# Autodesk Inventor assembly: XY Joint-Unit [B]
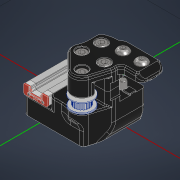
[picture p0: Inventor's stored thumbnail of the model, 180x180]
Saved by Autodesk Inventor 2022.2 (Build 262287010, 287A)
## iProperties
Created: 2022-03-15
Part Number: XY Joint-Unit [B]
Document SubType Name: Assembly
Designer: sleib
Author: sleib
## Documents named in this file (11)
- C:\Users\sleib\Projekte\Voron-2\CAD\Inventor\XY Joint-Unit [B].iam
- C:\Users\sleib\Projekte\Voron-2\CAD\Inventor\M3x16 SHCS.ipt
- C:\Users\sleib\Projekte\Voron-2\CAD\Inventor\MGN9H Carriage.ipt
- C:\Users\sleib\Projekte\Voron-2\CAD\Inventor\M5x40 SHCS.ipt
- C:\Users\sleib\Projekte\Voron-2\CAD\Inventor\M5 Hexnut.ipt
- C:\Users\sleib\Projekte\Voron-2\CAD\Inventor\GT2 20T Idler (6mm).ipt
- C:\Users\sleib\Projekte\Voron-2\CAD\Inventor\M5 Spacer (1mm).ipt
- C:\Users\sleib\Projekte\Voron-2\CAD\Inventor\Bearing F695-ZZ.ipt
- C:\Users\sleib\Projekte\Voron-2\CAD\Inventor\M5x30 BHCS.ipt
- C:\Users\sleib\Projekte\Voron-2\CAD\Inventor\M5x10 BHCS.ipt
- C:\Users\sleib\Projekte\Voron-2\CAD\Inventor\XY Joint MGN12H [B].ipt
## Components (21 placed, 10 different names)
1. XY Joint MGN12H [B]:1 — Fluchtend:1, Passend:42, Passend:43, Passend:44, Passend:45, Passend:46, Passend:47, Passend:48, Passend:49, Passend:50, Passend:51, Passend:52, Passend:53, Passend:54, Passend:55, Winkel:1, Passend:56, Passend:57, Winkel:2, Passend:58, Passend:59, Passend:60, Passend:61, Passend:62, Passend:63, Passend:64, Passend:65, Passend:66, Passend:67, Passend:68, Passend:69, Winkel:3, Passend:70, Passend:71
2. MGN9H Carriage:1 — Passend:49, Passend:72, Passend:73, Passend:74, Passend:75
3. GT2 20T Idler (6mm):1 — Passend:30, Passend:69
4. Bearing F695-ZZ:1 — Passend:34, Passend:38, Passend:39
5. Bearing F695-ZZ:2 — Passend:35, Passend:37, Passend:39
6. M3x16 SHCS:1 — Passend:45, Passend:52, Passend:72
7. M3x16 SHCS:2 — Passend:47, Passend:51, Passend:75
8. M3x16 SHCS:3 — Passend:48, Passend:50, Passend:73
9. M3x16 SHCS:4 — Passend:46, Passend:53, Passend:74
10. M5x40 SHCS:1 — Passend:24, Passend:71
11. M5x40 SHCS:2 — Passend:23, Passend:33, Passend:34, Passend:35, Passend:36, Passend:41
12. M5x40 SHCS:3 — Passend:30, Passend:67, Passend:68
13. M5x40 SHCS:4 — Passend:22, Passend:60
14. M5 Hexnut:1 — Passend:23, Passend:54, Winkel:1, Passend:56
15. M5 Hexnut:2 — Passend:24, Passend:59, Winkel:3, Passend:70
16. M5 Hexnut:3 — Passend:22, Passend:57, Winkel:2, Passend:58
17. M5 Spacer (1mm):1 — Passend:33, Passend:38, Passend:41
18. M5 Spacer (1mm):2 — Passend:36, Passend:37, Passend:55
19. M5x30 BHCS:1 — Passend:65, Passend:66
20. M5x10 BHCS:1 — Passend:62, Passend:64
21. M5x10 BHCS:2 — Passend:61, Passend:63
## Relationships (50: Mate 46, Angle 3, Flush 1)
- Passend:22 [Mate]: M5x40 SHCS:4 ↔ M5 Hexnut:3
- Passend:23 [Mate]: M5x40 SHCS:2 ↔ M5 Hexnut:1
- Passend:24 [Mate]: M5x40 SHCS:1 ↔ M5 Hexnut:2
- Passend:30 [Mate]: GT2 20T Idler (6mm):1 ↔ M5x40 SHCS:3
- Passend:33 [Mate]: M5x40 SHCS:2 ↔ M5 Spacer (1mm):1
- Passend:34 [Mate]: Bearing F695-ZZ:1 ↔ M5x40 SHCS:2
- Passend:35 [Mate]: Bearing F695-ZZ:2 ↔ M5x40 SHCS:2
- Passend:36 [Mate]: M5x40 SHCS:2 ↔ M5 Spacer (1mm):2
- Passend:37 [Mate]: Bearing F695-ZZ:2 ↔ M5 Spacer (1mm):2
- Passend:38 [Mate]: Bearing F695-ZZ:1 ↔ M5 Spacer (1mm):1
- Passend:39 [Mate]: Bearing F695-ZZ:1 ↔ Bearing F695-ZZ:2
- Passend:41 [Mate]: M5x40 SHCS:2 ↔ M5 Spacer (1mm):1
- Fluchtend:1 [Flush]: XY Joint MGN12H [B]:1
- Passend:42 [Mate]: XY Joint MGN12H [B]:1
- Passend:43 [Mate]: XY Joint MGN12H [B]:1
- Passend:44 [Mate] (-7.5 mm): XY Joint MGN12H [B]:1
- Passend:45 [Mate]: XY Joint MGN12H [B]:1 ↔ M3x16 SHCS:1
- Passend:46 [Mate]: XY Joint MGN12H [B]:1 ↔ M3x16 SHCS:4
- Passend:47 [Mate]: XY Joint MGN12H [B]:1 ↔ M3x16 SHCS:2
- Passend:48 [Mate]: XY Joint MGN12H [B]:1 ↔ M3x16 SHCS:3
- Passend:49 [Mate]: XY Joint MGN12H [B]:1 ↔ MGN9H Carriage:1
- Passend:50 [Mate]: XY Joint MGN12H [B]:1 ↔ M3x16 SHCS:3
- Passend:51 [Mate]: XY Joint MGN12H [B]:1 ↔ M3x16 SHCS:2
- Passend:52 [Mate]: XY Joint MGN12H [B]:1 ↔ M3x16 SHCS:1
- Passend:53 [Mate]: XY Joint MGN12H [B]:1 ↔ M3x16 SHCS:4
- Passend:54 [Mate]: XY Joint MGN12H [B]:1 ↔ M5 Hexnut:1
- Passend:55 [Mate]: XY Joint MGN12H [B]:1 ↔ M5 Spacer (1mm):2
- Winkel:1 [Angle] (0 deg): XY Joint MGN12H [B]:1 ↔ M5 Hexnut:1
- Passend:56 [Mate]: XY Joint MGN12H [B]:1 ↔ M5 Hexnut:1
- Passend:57 [Mate]: XY Joint MGN12H [B]:1 ↔ M5 Hexnut:3
- Winkel:2 [Angle] (0 deg): XY Joint MGN12H [B]:1 ↔ M5 Hexnut:3
- Passend:58 [Mate]: XY Joint MGN12H [B]:1 ↔ M5 Hexnut:3
- Passend:59 [Mate]: XY Joint MGN12H [B]:1 ↔ M5 Hexnut:2
- Passend:60 [Mate]: XY Joint MGN12H [B]:1 ↔ M5x40 SHCS:4
- Passend:61 [Mate]: XY Joint MGN12H [B]:1 ↔ M5x10 BHCS:2
- Passend:62 [Mate]: XY Joint MGN12H [B]:1 ↔ M5x10 BHCS:1
- Passend:63 [Mate]: XY Joint MGN12H [B]:1 ↔ M5x10 BHCS:2
- Passend:64 [Mate]: XY Joint MGN12H [B]:1 ↔ M5x10 BHCS:1
- Passend:65 [Mate]: XY Joint MGN12H [B]:1 ↔ M5x30 BHCS:1
- Passend:66 [Mate]: XY Joint MGN12H [B]:1 ↔ M5x30 BHCS:1
- Passend:67 [Mate]: XY Joint MGN12H [B]:1 ↔ M5x40 SHCS:3
- Passend:68 [Mate]: XY Joint MGN12H [B]:1 ↔ M5x40 SHCS:3
- Passend:69 [Mate]: XY Joint MGN12H [B]:1 ↔ GT2 20T Idler (6mm):1
- Winkel:3 [Angle] (0 deg): XY Joint MGN12H [B]:1 ↔ M5 Hexnut:2
- Passend:70 [Mate]: XY Joint MGN12H [B]:1 ↔ M5 Hexnut:2
- Passend:71 [Mate]: XY Joint MGN12H [B]:1 ↔ M5x40 SHCS:1
- Passend:72 [Mate]: MGN9H Carriage:1 ↔ M3x16 SHCS:1
- Passend:73 [Mate]: MGN9H Carriage:1 ↔ M3x16 SHCS:3
- Passend:74 [Mate]: MGN9H Carriage:1 ↔ M3x16 SHCS:4
- Passend:75 [Mate]: MGN9H Carriage:1 ↔ M3x16 SHCS:2
